# Autodesk Inventor assembly: 10-CJ2B10-15RZ(0_1_0)
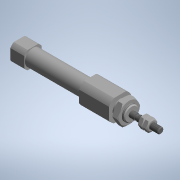
[picture p0: Inventor's stored thumbnail of the model, 180x180]
Saved by Autodesk Inventor 2022.3 (Build 263350000, 350)
## iProperties
Category: PARTsolutions
Company: SMC
Part Number: 10-CJ2B10-15RZ(0_1_0)
Catalog Web Link: www.cadenas.de
Description: 10/11-CJ2-Z/10/11-CDJ2-Z-Air Cylinder/Standard: Double Acting Single Rod/Clean Series
Vendor: SMC
Document SubType Name: Assembly
Designer: partserver
Manufacturer: SMC
Mass: 9.46733 g
Surface Area: 67.6244 cm^2
Volume: 9.46733 cm^3
PSOL_IDENT_0: {$CADENAS_DATA\23d-libs\smc_jp\actuator\standard_air_cylinder\cj2\10_cj2_z_asmtab.prj},297 {VTYP=3D}
PSOL_IDENT_1: ,{STYP=ASSTAB},{NB=10-CJ2B10-15RZ(0_1_0)},{LINA=10-CJ2B10-15RZ},{NN=10/11-CJ2-Z/10/11-CDJ2-Z},{DATE=
PSOL_IDENT_2: 17.11.2021 19:03:25},{GEOMDATE=08.04.2020 08:30:03},{VERSION=},{LINEID=370},{WBVAR=TYPE,MAGNET,AUTOS
PSOL_IDENT_3: WITCH,LEAD,NUMBER,CUSHION,STROKE,POS,PORT,STOP,MOUNTING,THREAD},{WBNUMERIC=STROKE,POS}  {NB=10-CJ2B1
PSOL_IDENT_4: 0-15RZ(0_1_0)},{LINA=10-CJ2B10-15RZ},{KT=DUMMY},{NENN=10-CJ2B10-15},{TYPE=10},{ORDER=10-CJ2B10-15RZ}
PSOL_IDENT_5: ,{BORE=10},{MOUNT=(B) Basic},{MOUNTX=B},{MAGNET=},{AUTOSWITCH=},{AUTOSWX='','N/A'},{LEAD=},{LEADX= ''
PSOL_IDENT_6: ,'N/A' },{NUMBER=},{CUSHION=},{CUSHIONX= '','(-) Rubber cushion','A','(A) Air cushion' },{SWSIGNX= ''
PSOL_IDENT_7: ,'N/A' },{STROKE=15},{STDSTROKE=15,30,45,60,75,100,125,150},{STROKE1X=[2:150/1]},{SMIN=2},{SMINASW1=
PSOL_IDENT_8: 10},{SMINASW2=15},{SMAX1=150},{POS=0},{PORT=R},{STOP=1},{COM=Please confirm the conditions of use wi
PSOL_IDENT_9: th SMC},{MOUNTING=},{THREAD=0},{MOUNTINGX='','N/A'},{PORTX='', '(-) Perpendicular', 'R', '(R) In-lin
PSOL_IDENT_10: e'},{SW=B},{PPATH=10_cj2_z/assembly/10_cj2_z_asmsbl.prj}
NB: 10-CJ2B10-15RZ(0_1_0)
NN: 10/11-CJ2-Z/10/11-CDJ2-Z
NT: Air Cylinder/Standard: Double Acting Single Rod/Clean Series
NBSYN: $ORDER.($POS._$STOP._$THREAD.)
LINA: 10-CJ2B10-15RZ
CATALOG: SMC (JP
TYPE: (10) Relief type
BORE: 10
MOUNT: (B) Basic
MAGNET: (-) Without magnet
AUTOSWITCH: N/A
LEAD: N/A
NUMBER: N/A
CUSHION: (-) Rubber cushion
STROKE: 15
POS: 0
PORT: (R) In-line
STOP: Manufacturable stroke
MOUNTING: N/A
THREAD: on
SUPPLIER: SMC
ARTICLENO: 10-CJ2B10-15RZ(0_1_0)
BOMINFO: 10-CJ2B10-15RZ
CREATOR: CADENAS GmbH
Title: 10-CJ2B10-15RZ
Author: Cadenas PARTsolutions
Comments: Air Cylinder/Standard: Double Acting Single Rod/Clean Series
## Documents named in this file (5)
- C:\Users\YusukeKunita\Documents\GrabCAD\Development\BasicParts\AirCylinder\10-CJ2B10-15RZ(0_1_0)\10-CJ2B10-15RZ.iam
- C:\Users\YusukeKunita\Documents\GrabCAD\Development\BasicParts\AirCylinder\10-CJ2B10-15RZ(0_1_0)\10-CJ2B10-15RZ_BODY.ipt
- C:\Users\YusukeKunita\Documents\GrabCAD\Development\BasicParts\AirCylinder\10-CJ2B10-15RZ(0_1_0)\10_11-CJ2B10-15Z_ROD.ipt
- C:\Users\YusukeKunita\Documents\GrabCAD\Development\BasicParts\AirCylinder\10-CJ2B10-15RZ(0_1_0)\NTJ-010A_CJ2.ipt
- C:\Users\YusukeKunita\Documents\GrabCAD\Development\BasicParts\AirCylinder\10-CJ2B10-15RZ(0_1_0)\10-CJ210Z_NUT.ipt
## Components (5 placed, 4 different names)
1. 10-CJ2B10-15RZ_BODY:1 — body_Z@1 <-> ROD_BODY_Z@2, body_YZ@1 <-> ROD_BODY_YZ@2, body_XY@1 <-> NUT_XY@5, body_Z@1 <-> NUT_Z@5, body_YZ@1 <-> NUT_YZ@5, フラッシュ:1
2. 10_11-CJ2B10-15Z_ROD:1 — body_Z@1 <-> ROD_BODY_Z@2, body_YZ@1 <-> ROD_BODY_YZ@2, rodnt1_XY@2 <-> nt_XY@3, rodnt1_Z@2 <-> nt_Z@3, rodnt1_YZ@2 <-> nt_YZ@3, rodnt1_XY@2 <-> nt_XY@4, rodnt1_Z@2 <-> nt_Z@4, rodnt1_YZ@2 <-> nt_YZ@4, フラッシュ:1
3. NTJ-010A_CJ2:1 — rodnt1_XY@2 <-> nt_XY@3, rodnt1_Z@2 <-> nt_Z@3, rodnt1_YZ@2 <-> nt_YZ@3
4. NTJ-010A_CJ2:2 — rodnt1_XY@2 <-> nt_XY@4, rodnt1_Z@2 <-> nt_Z@4, rodnt1_YZ@2 <-> nt_YZ@4
5. 10-CJ210Z_NUT:1 — body_XY@1 <-> NUT_XY@5, body_Z@1 <-> NUT_Z@5, body_YZ@1 <-> NUT_YZ@5
## Relationships (12: Mate 7, Angle 4, Flush 1)
- body_Z@1 <-> ROD_BODY_Z@2 [Mate]: 10-CJ2B10-15RZ_BODY:1 ↔ 10_11-CJ2B10-15Z_ROD:1
- body_YZ@1 <-> ROD_BODY_YZ@2 [Angle] (0 deg): 10-CJ2B10-15RZ_BODY:1 ↔ 10_11-CJ2B10-15Z_ROD:1
- rodnt1_XY@2 <-> nt_XY@3 [Mate]: 10_11-CJ2B10-15Z_ROD:1 ↔ NTJ-010A_CJ2:1
- rodnt1_Z@2 <-> nt_Z@3 [Mate]: 10_11-CJ2B10-15Z_ROD:1 ↔ NTJ-010A_CJ2:1
- rodnt1_YZ@2 <-> nt_YZ@3 [Angle] (0 deg): 10_11-CJ2B10-15Z_ROD:1 ↔ NTJ-010A_CJ2:1
- rodnt1_XY@2 <-> nt_XY@4 [Mate] (3.2 mm): 10_11-CJ2B10-15Z_ROD:1 ↔ NTJ-010A_CJ2:2
- rodnt1_Z@2 <-> nt_Z@4 [Mate]: 10_11-CJ2B10-15Z_ROD:1 ↔ NTJ-010A_CJ2:2
- rodnt1_YZ@2 <-> nt_YZ@4 [Angle] (0 deg): 10_11-CJ2B10-15Z_ROD:1 ↔ NTJ-010A_CJ2:2
- body_XY@1 <-> NUT_XY@5 [Mate] (-2.3 mm): 10-CJ2B10-15RZ_BODY:1 ↔ 10-CJ210Z_NUT:1
- body_Z@1 <-> NUT_Z@5 [Mate]: 10-CJ2B10-15RZ_BODY:1 ↔ 10-CJ210Z_NUT:1
- body_YZ@1 <-> NUT_YZ@5 [Angle] (0 deg): 10-CJ2B10-15RZ_BODY:1 ↔ 10-CJ210Z_NUT:1
- フラッシュ:1 [Flush]: 10-CJ2B10-15RZ_BODY:1 ↔ 10_11-CJ2B10-15Z_ROD:1
